# Autodesk Inventor assembly: GE-11041
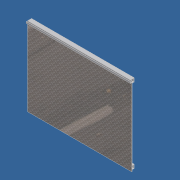
[picture p0: Inventor's stored thumbnail of the model, 180x180]
Saved by Autodesk Inventor 2012 (Build 160160000, 160)
## iProperties
Created: 2010-09-30
Part Number: GE-11041
Document SubType Name: Assembly
Designer: mcyr
Author: mcyr
## Documents named in this file (7)
- C:\Data Folder\FRC 2012 Field\Components\GE-11041r.iam
- C:\Data Folder\FRC 2012 Field\Components\Velcro.ipt
- C:\Data Folder\FRC 2012 Field\Components\GE-11041-02.ipt
- C:\Data Folder\FRC 2012 Field\Components\GE-11041-03.ipt
- C:\Data Folder\FRC 2012 Field\Components\GE-11041-04.ipt
- C:\Data Folder\FRC 2012 Field\Components\GE-11041-01.ipt
- C:\Data Folder\FRC 2012 Field\Components\GE-11041-05.iam
## Components (9 placed, 6 different names)
1. GE-11041-02:1 — Flush:10, Mate:13, Flush:19
2. GE-11041-03:1 — Mate:8, Flush:12, Flush:13, Mate:13, Flush:19
3. GE-11041-03:2 — Mate:9, Flush:14, Mate:10, Mate:11, Flush:16, Flush:20, Mate:16
4. GE-11041-04:1 — Mate:6, Flush:8, Flush:9, Mate:12, Flush:17, Flush:18, Mate:14, Flush:21, Flush:22
5. Velcro:1 — Mate:6, Flush:8, Flush:9
6. GE-11041-01:1 — Flush:10, Mate:8, Flush:12, Flush:13, Mate:9, Flush:14, Flush:20, Mate:15, Flush:23
7. GE-11041-05:1 [sub-assembly] — Mate:10, Mate:11, Flush:16, Mate:12, Flush:17, Flush:18
8. Velcro:2 — Mate:15, Mate:16, Flush:23
9. Velcro:3 — Mate:14, Flush:21, Flush:22
## Relationships (24: Flush 14, Mate 10)
- Mate:6: GE-11041-04:1 ↔ Velcro:1
- Flush:8: GE-11041-04:1 ↔ Velcro:1
- Flush:9: GE-11041-04:1 ↔ Velcro:1
- Flush:10: GE-11041-02:1 ↔ GE-11041-01:1
- Mate:8: GE-11041-03:1 ↔ GE-11041-01:1
- Flush:12 (19.05 mm): GE-11041-03:1 ↔ GE-11041-01:1
- Flush:13 (-19.05 mm): GE-11041-03:1 ↔ GE-11041-01:1
- Mate:9: GE-11041-03:2 ↔ GE-11041-01:1
- Flush:14: GE-11041-03:2 ↔ GE-11041-01:1
- Mate:10: GE-11041-03:2 ↔ GE-11041-05:1
- Mate:11: GE-11041-03:2 ↔ GE-11041-05:1
- Flush:16 (405.638 mm): GE-11041-03:2 ↔ GE-11041-05:1
- Mate:12: GE-11041-04:1 ↔ GE-11041-05:1
- Flush:17: GE-11041-04:1 ↔ GE-11041-05:1
- Flush:18: GE-11041-04:1 ↔ GE-11041-05:1
- Mate:13: GE-11041-02:1 ↔ GE-11041-03:1
- Flush:19: GE-11041-02:1 ↔ GE-11041-03:1
- Flush:20: GE-11041-03:2 ↔ GE-11041-01:1
- Mate:14: GE-11041-04:1 ↔ Velcro:3
- Flush:21: GE-11041-04:1 ↔ Velcro:3
- Flush:22: GE-11041-04:1 ↔ Velcro:3
- Mate:15: GE-11041-01:1 ↔ Velcro:2
- Mate:16 (209.55 mm): GE-11041-03:2 ↔ Velcro:2
- Flush:23 (415.925 mm): GE-11041-01:1 ↔ Velcro:2
